# Autodesk Inventor assembly: TwinsChamberAndCoils
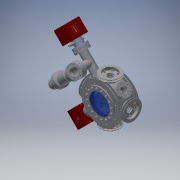
[picture p0: Inventor's stored thumbnail of the model, 180x180]
Saved by Autodesk Inventor 2016 (Build 200138000, 138)
## iProperties
Created: 2015-05-05
Part Number: TwinsChamberAndCoils
Document SubType Name: Assembly
Designer: MG
Author: MG
## Documents named in this file (4)
- C:\Users\Michael\Dropbox (Personal)\Code\CAD---Experiment-systems\twins\Chamber\TwinsChamberAndCoils.iam
- C:\Users\Michael\Dropbox (MIT)\Quanta\MG\CAD\Experiment\Twins\MainChamber_wTwinCavity.iam
- C:\Users\Michael\Dropbox (MIT)\Quanta\MG\CAD\BfieldCoils\TwinsBfieldASM.iam
- C:\Users\Michael\Dropbox (Personal)\DO_NOT_DELETE\Flanges\Windows\VPZL-275Q.iam
## Components (3 placed, 3 different names)
1. MainChamber_wTwinCavity:1 [sub-assembly] — Angle:2, Insert:13, Insert:14
2. TwinsBfieldASM:1 [sub-assembly] — Angle:2, Insert:13
3. VPZL-275Q:1 [sub-assembly] — Insert:14
## Relationships (3: Insert 2, Angle 1)
- Angle:2 (0 deg): MainChamber_wTwinCavity:1 ↔ TwinsBfieldASM:1
- Insert:13: MainChamber_wTwinCavity:1 ↔ TwinsBfieldASM:1
- Insert:14: MainChamber_wTwinCavity:1 ↔ VPZL-275Q:1
